# Autodesk Inventor assembly: Gimbal_IMU_Sled_Assembly
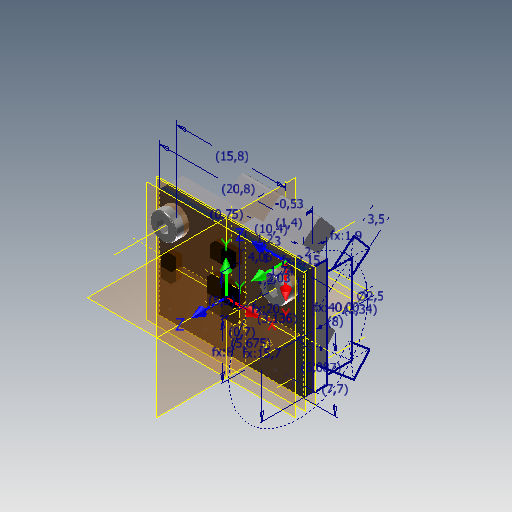
[picture p0: Inventor's stored thumbnail of the model, 512x512]
Saved by Autodesk Inventor 2021.4 (Build 254397000, 397)
## iProperties
Created: 2022-08-24
Part Number: Gimbal_IMU_Sled_Assembly
Material: Generisch
Document SubType Name: Assembly
Designer: alexw
Mass: 2.28207 g
Surface Area: 21.0816 cm^2
Volume: 1.84118 cm^3
Density: 1.23946 g/cm^3
Author: alexw
## Documents named in this file (5)
- C:\Users\alexw\Documents\Inventor\Projects\03_CurrentProjects\MasterThesis\TrainingConsol_220422\Workgroups\Workgroup\Gimbal_IMU_Sled_Assembly.iam
- C:\Users\alexw\Documents\Inventor\Projects\03_CurrentProjects\MasterThesis\TrainingConsol_220422\Workgroups\Workgroup_new\IMU_Fixation.ipt
- C:\Users\alexw\Documents\Inventor\Projects\03_CurrentProjects\MasterThesis\TrainingConsol_220422\Workgroups\Workgroup\ContentCenter\en-US\ISO 4762(2)\ISO 4762 - M2 x 4ISO.ipt
- C:\Users\alexw\Documents\Inventor\Projects\03_CurrentProjects\MasterThesis\TrainingConsol_220422\Workgroups\Workgroup_new\GY_521_v2.iam
- C:\Users\alexw\Documents\Inventor\Projects\03_CurrentProjects\MasterThesis\TrainingConsol_220422\Workgroups\Workgroup\HallEffectSensor.ipt
## Components (5 placed, 4 different names)
1. IMU_Fixation:1 — Mate:7, Mate:11, Mate:13, Flush:3, Mate:19, Mate:21
2. ISO 4762 M2 x 4:1 — Mate:7, Mate:15, Mate:16
3. ISO 4762 M2 x 4:3 — Mate:11, Mate:12, Mate:14
4. GY_521_v2:1 [sub-assembly] — Mate:12, Mate:13, Flush:1, Flush:2, Mate:14, Mate:15, Mate:16, Angle:1, Mate:17
5. HallEffectSensor:1 — Angle:1, Mate:17, Angle:2, Mate:20, Mate:21
## Relationships (16: Mate 11, Flush 3, Angle 2)
- Mate:7: IMU_Fixation:1 ↔ ISO 4762 M2 x 4:1
- Mate:11: IMU_Fixation:1 ↔ ISO 4762 M2 x 4:3
- Mate:12: ISO 4762 M2 x 4:3 ↔ GY_521_v2:1
- Mate:13: IMU_Fixation:1 ↔ GY_521_v2:1
- Flush:1: GY_521_v2:1
- Flush:2: GY_521_v2:1
- Flush:3: IMU_Fixation:1
- Mate:14: ISO 4762 M2 x 4:3 ↔ GY_521_v2:1
- Mate:15: ISO 4762 M2 x 4:1 ↔ GY_521_v2:1
- Mate:16: ISO 4762 M2 x 4:1 ↔ GY_521_v2:1
- Angle:1 (0 deg): GY_521_v2:1 ↔ HallEffectSensor:1
- Mate:17: GY_521_v2:1 ↔ HallEffectSensor:1
- Mate:19: IMU_Fixation:1
- Angle:2 (0 deg): HallEffectSensor:1
- Mate:20: HallEffectSensor:1
- Mate:21: IMU_Fixation:1 ↔ HallEffectSensor:1
